# Autodesk Inventor assembly: motherboard_gpu
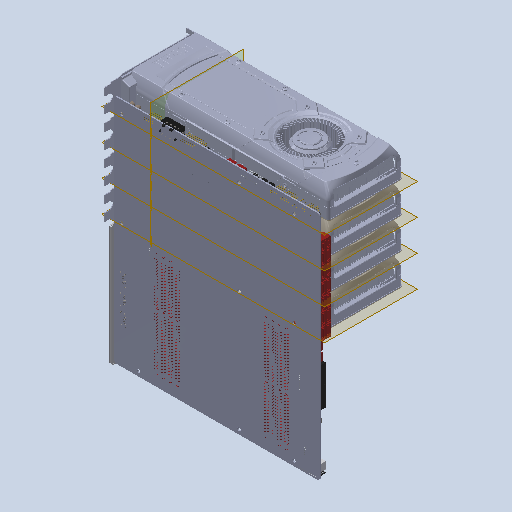
[picture p0: Inventor's stored thumbnail of the model, 512x512]
Saved by Autodesk Inventor 2022 (Build 260153000, 153)
## iProperties
Created: 2021-05-09
Part Number: motherboard_gpu
Document SubType Name: Assembly
Designer: gisen
Author: gisen
## Documents named in this file (3)
- C:\Users\gisen\Documents\GitHub\eatx_case\atx\resources\motherboard_gpu.iam
- C:\Users\gisen\Documents\GitHub\eatx_case\atx\resources\motherboard\Rampage V Extreme Assembly.iam
- C:\Users\gisen\Documents\GitHub\eatx_case\atx\resources\gpu\titan assembly.iam
## Components (5 placed, 2 different names)
1. Rampage V Extreme Assembly:1 [sub-assembly] — Flush:1, Mate:1, Flush:2, Mate:2, Flush:5, Flush:6, Mate:3, Flush:9, Mate:4
2. titan assembly:1 [sub-assembly] — Flush:1, Mate:1, Flush:2, Flush:4, Flush:7, Flush:8
3. titan assembly:2 [sub-assembly] — Flush:4, Mate:2, Flush:5
4. titan assembly:3 [sub-assembly] — Flush:6, Flush:7, Mate:3
5. titan assembly:4 [sub-assembly] — Flush:8, Flush:9, Mate:4
## Relationships (12: Flush 8, Mate 4)
- Flush:1 (-109.72 mm): Rampage V Extreme Assembly:1 ↔ titan assembly:1
- Mate:1: Rampage V Extreme Assembly:1 ↔ titan assembly:1
- Flush:2: Rampage V Extreme Assembly:1 ↔ titan assembly:1
- Flush:4: titan assembly:1 ↔ titan assembly:2
- Mate:2: Rampage V Extreme Assembly:1 ↔ titan assembly:2
- Flush:5: Rampage V Extreme Assembly:1 ↔ titan assembly:2
- Flush:6: Rampage V Extreme Assembly:1 ↔ titan assembly:3
- Flush:7: titan assembly:1 ↔ titan assembly:3
- Mate:3: Rampage V Extreme Assembly:1 ↔ titan assembly:3
- Flush:8: titan assembly:1 ↔ titan assembly:4
- Flush:9: Rampage V Extreme Assembly:1 ↔ titan assembly:4
- Mate:4: Rampage V Extreme Assembly:1 ↔ titan assembly:4
